# Autodesk Inventor assembly: armasembaly2
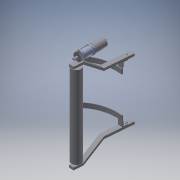
[picture p0: Inventor's stored thumbnail of the model, 180x180]
Saved by Autodesk Inventor 2016 (Build 200138000, 138)
## iProperties
Created: 2016-01-18
Part Number: armasembaly2
Document SubType Name: Assembly
Designer: Thariq
Author: Thariq
## Documents named in this file (10)
- C:\Users\Thariq\Documents\armasembaly2.iam
- C:\Users\Thariq\Documents\arm2.ipt
- C:\Users\Thariq\Documents\axel.ipt
- C:\Users\Thariq\Documents\roller.ipt
- C:\Users\Thariq\Documents\rail.ipt
- C:\Users\Thariq\Documents\connector1by1.ipt
- C:\Users\Thariq\Documents\1by225connector.ipt
- C:\Users\Thariq\Documents\am-2877+Banebots+P60+64-1.ipt
- C:\Users\Thariq\Documents\217-4347-STEP-20141030.ipt
- C:\Users\Thariq\Documents\am-2631+32T+20dp+10mmk.ipt
## Components (13 placed, 9 different names)
1. arm2:1 — Mate:1, Flush:1, Flush:2, Mate:2, Mate:3, Flush:3, Mate:8, Mate:9, Flush:5, Flush:7, Mate:17
2. arm2:2 — Mate:1, Flush:1, Flush:2, Mate:11, Flush:6, Flush:9, Flush:11, Mate:16
3. axel:1 — Mate:2, Mate:3, Mate:4, Mate:5, Mate:6, Flush:11, Mate:15, Mate:16
4. roller:1 — Mate:4, Mate:15, Mate:17
5. rail:1 — Mate:6, Flush:3, Flush:4, Mate:7, Mate:8, Mate:10, Flush:8
6. rail:2 — Mate:5, Flush:4, Mate:7, Mate:12, Flush:10, Mate:14
7. connector1by1:1 — Mate:9, Mate:10, Flush:5, Mate:13
8. connector1by1:2 — Mate:11, Flush:6, Mate:12
9. 1by225connector:1 — Mate:13, Flush:7, Flush:8
10. 1by225connector:2 — Flush:9, Flush:10, Mate:14
11. am-2877+Banebots+P60+64-1:1 — Mate:18, Mate:19, Mate:20
12. 217-4347-STEP-20141030:1 — Mate:18, Mate:19
13. am-2631+32T+20dp+10mmk:1 — Mate:20
## Relationships (31: Mate 20, Flush 11)
- Mate:1 (304.8 mm): arm2:1 ↔ arm2:2
- Flush:1: arm2:1 ↔ arm2:2
- Flush:2: arm2:1 ↔ arm2:2
- Mate:2: arm2:1 ↔ axel:1
- Mate:3: arm2:1 ↔ axel:1
- Mate:4: axel:1 ↔ roller:1
- Mate:5: axel:1 ↔ rail:2
- Mate:6: axel:1 ↔ rail:1
- Flush:3 (12.7 mm): arm2:1 ↔ rail:1
- Flush:4: rail:1 ↔ rail:2
- Mate:7 (190.5 mm): rail:1 ↔ rail:2
- Mate:8 (31.75 mm): arm2:1 ↔ rail:1
- Mate:9: arm2:1 ↔ connector1by1:1
- Mate:10 (3.175 mm): rail:1 ↔ connector1by1:1
- Flush:5: arm2:1 ↔ connector1by1:1
- Mate:11: arm2:2 ↔ connector1by1:2
- Flush:6: arm2:2 ↔ connector1by1:2
- Mate:12 (3.175 mm): rail:2 ↔ connector1by1:2
- Mate:13: connector1by1:1 ↔ 1by225connector:1
- Flush:7: arm2:1 ↔ 1by225connector:1
- Flush:8: rail:1 ↔ 1by225connector:1
- Flush:9: arm2:2 ↔ 1by225connector:2
- Flush:10: rail:2 ↔ 1by225connector:2
- Mate:14: rail:2 ↔ 1by225connector:2
- Flush:11: arm2:2 ↔ axel:1
- Mate:15: axel:1 ↔ roller:1
- Mate:16: arm2:2 ↔ axel:1
- Mate:17 (3.175 mm): arm2:1 ↔ roller:1
- Mate:18: am-2877+Banebots+P60+64-1:1 ↔ 217-4347-STEP-20141030:1
- Mate:19: am-2877+Banebots+P60+64-1:1 ↔ 217-4347-STEP-20141030:1
- Mate:20: am-2877+Banebots+P60+64-1:1 ↔ am-2631+32T+20dp+10mmk:1
